# Autodesk Inventor assembly: fullArm
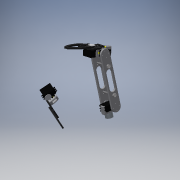
[picture p0: Inventor's stored thumbnail of the model, 180x180]
Saved by Autodesk Inventor 2016 (Build 200138000, 138)
## iProperties
Created: 2015-10-07
Part Number: fullArm
Document SubType Name: Assembly
Designer: alex
Author: alex
## Documents named in this file (8)
- C:\Users\alex\Workspace\arm\CAD\fullArm.iam
- C:\Users\alex\Workspace\arm\CAD\ArmBase.ipt
- C:\Users\alex\Workspace\arm\CAD\LowerArm.ipt
- C:\Users\alex\Workspace\arm\CAD\servo.ipt
- C:\Users\alex\Documents\Inventor\Content Center Files\R2016\en-US\AS 1427(02)\AS 1427 - M8 x 65(2).ipt
- C:\Users\alex\Workspace\arm\CAD\GripperAttachment.ipt
- C:\Users\alex\Workspace\arm\CAD\stepperMotor.ipt
- C:\Users\alex\Workspace\arm\CAD\Claw.ipt
## Components (15 placed, 7 different names)
1. LowerArm:1 — Rotational:3, Cylindrical:1, Cylindrical:2, Mate:5, Rotational:4, Rigid:2, Rotational:5
2. LowerArm:2 — Mate:1, Mate:2, Mate:3, Mate:4
3. servo:1 — Mate:9, Mate:10, Mate:11, Rotational:5
4. servo:2 — Rotational:3, Mate:6, Mate:7, Mate:8
5. AS 1427 - Metric M8 x 65:1 — Mate:1, Mate:2, Cylindrical:1, Mate:5, Rotational:4
6. AS 1427 - Metric M8 x 65:2 — Mate:3, Mate:4, Cylindrical:2, Rigid:2
7. GripperAttachment:1 — Mate:6, Mate:7, Mate:8, Mate:12, Mate:13, Mate:17
8. ArmBase:1 — Mate:9, Mate:10, Mate:11, Mate:18
9. stepperMotor:2 — Mate:18
10. Claw:1 — Mate:12, Mate:13, Mate:14, Mate:15, Mate:16, Mate:17
11. servo:3 — Mate:14, Mate:15, Mate:16
12. GripperAttachment:2 — Mate:19, Mate:20, Mate:21, Mate:22, Mate:23
13. servo:4
14. servo:5 — Mate:19, Mate:20, Mate:21
15. Claw:2 — Mate:22, Mate:23
## Relationships (29: Mate 23, RevoluteJoint 3, CylindricalJoint 2, WeldJoint 1)
- Rotational:3 [RevoluteJoint]: LowerArm:1 ↔ servo:2
- Mate:1: LowerArm:2 ↔ AS 1427 - Metric M8 x 65:1
- Mate:2: LowerArm:2 ↔ AS 1427 - Metric M8 x 65:1
- Mate:3: LowerArm:2 ↔ AS 1427 - Metric M8 x 65:2
- Mate:4: LowerArm:2 ↔ AS 1427 - Metric M8 x 65:2
- Cylindrical:1: LowerArm:1 ↔ AS 1427 - Metric M8 x 65:1
- Cylindrical:2: LowerArm:1 ↔ AS 1427 - Metric M8 x 65:2
- Mate:5: LowerArm:1 ↔ AS 1427 - Metric M8 x 65:1
- Rotational:4 [RevoluteJoint]: LowerArm:1 ↔ AS 1427 - Metric M8 x 65:1
- Rigid:2 [WeldJoint]: LowerArm:1 ↔ AS 1427 - Metric M8 x 65:2
- Mate:6: servo:2 ↔ GripperAttachment:1
- Mate:7: servo:2 ↔ GripperAttachment:1
- Mate:8: servo:2 ↔ GripperAttachment:1
- Mate:9: servo:1 ↔ ArmBase:1
- Mate:10: servo:1 ↔ ArmBase:1
- Mate:11: servo:1 ↔ ArmBase:1
- Mate:12: GripperAttachment:1 ↔ Claw:1
- Mate:13: GripperAttachment:1 ↔ Claw:1
- Mate:14: Claw:1 ↔ servo:3
- Mate:15: Claw:1 ↔ servo:3
- Mate:16: Claw:1 ↔ servo:3
- Mate:17: GripperAttachment:1 ↔ Claw:1
- Rotational:5 [RevoluteJoint]: LowerArm:1 ↔ servo:1
- Mate:18: ArmBase:1 ↔ stepperMotor:2
- Mate:19: GripperAttachment:2 ↔ servo:5
- Mate:20: GripperAttachment:2 ↔ servo:5
- Mate:21: GripperAttachment:2 ↔ servo:5
- Mate:22: GripperAttachment:2 ↔ Claw:2
- Mate:23: GripperAttachment:2 ↔ Claw:2
